# Autodesk Inventor assembly: Body
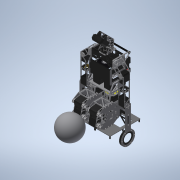
[picture p0: Inventor's stored thumbnail of the model, 180x180]
Saved by Autodesk Inventor 2020.4 (Build 244396000, 396)
## iProperties
Created: 2021-09-30
Part Number: Body
Document SubType Name: Assembly
Designer: Masato Kubotera
Mass: 3144.39 g
Surface Area: 11186.7 cm^2
Volume: 1959.41 cm^3
Density: 1.60477 g/cm^3
Author: Masato Kubotera
## Documents named in this file (4)
- C:\Users\Masato\Documents\Inventor\CIT Brains_Inventor\OpenPlatform_ver3_0 - ve4_1 branch\Body.iam
- C:\Users\Masato\Documents\Inventor\CIT Brains_Inventor\OpenPlatform_ver3_0 - ve4_1 branch\UpperBody\UpperBody.iam
- C:\Users\Masato\Documents\Inventor\CIT Brains_Inventor\OpenPlatform_ver3_0 - ve4_1 branch\LowerBody\LowerBody.iam
- C:\Users\Masato\Documents\Inventor\CIT Brains_Inventor\OpenPlatform_ver3_0 - ve4_1 branch\Ready_Made\Ball.ipt
## Components (4 placed, 3 different names)
1. Ball:1 — 正接:1, メイト:1, メイト:2
2. LowerBody:1 [sub-assembly] — メイト:3, フラッシュ:1, 角度:1, 挿入:1, 角度:2
3. LowerBody:2 [sub-assembly] — 角度:1, 挿入:2
4. UpperBody:1 [sub-assembly] — 挿入:1, 挿入:2, 角度:2, フラッシュ:2
## Relationships (10: Mate 3, Flush 2, Angle 2, Insert 2, Tangent 1)
- 正接:1 [Tangent]: Ball:1
- メイト:1 [Mate]: Ball:1
- メイト:2 [Mate]: Ball:1
- メイト:3 [Mate]: LowerBody:1
- フラッシュ:1 [Flush] (-200 mm): LowerBody:1
- 角度:1 [Angle] (0 deg): LowerBody:1 ↔ LowerBody:2
- 挿入:1 [Insert]: LowerBody:1 ↔ UpperBody:1
- 挿入:2 [Insert]: LowerBody:2 ↔ UpperBody:1
- 角度:2 [Angle] (0 deg): LowerBody:1 ↔ UpperBody:1
- フラッシュ:2 [Flush]: UpperBody:1
